# Autodesk Inventor assembly: scara 2.0
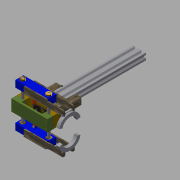
[picture p0: Inventor's stored thumbnail of the model, 180x180]
Saved by Autodesk Inventor 2019 (Build 230136000, 136)
## iProperties
Created: 2021-10-30
Part Number: scara 2.0
Document SubType Name: Assembly
Designer: Mohamed
Author: Mohamed
## Documents named in this file (21)
- F:\Semester 7\Design of mechatronics 1\SSCARA Robot\scara 2.0.iam
- F:\Semester 7\Design of mechatronics 1\SSCARA Robot\g_6mm rod.ipt
- F:\Semester 7\Design of mechatronics 1\SSCARA Robot\g_servo mount 1.ipt
- F:\Semester 7\Design of mechatronics 1\SSCARA Robot\g_servo mount 2.ipt
- F:\Semester 7\Design of mechatronics 1\SSCARA Robot\MG995.ipt
- F:\Semester 7\Design of mechatronics 1\SSCARA Robot\g_servo horn.ipt
- F:\Semester 7\Design of mechatronics 1\SSCARA Robot\g_connector x4.ipt
- F:\Semester 7\Design of mechatronics 1\SSCARA Robot\g_bolt.ipt
- F:\Semester 7\Design of mechatronics 1\SSCARA Robot\g_nut.ipt
- F:\Semester 7\Design of mechatronics 1\SSCARA Robot\g_griper side.ipt
- F:\Semester 7\Design of mechatronics 1\SSCARA Robot\g_griper side2.ipt
- F:\Semester 7\Design of mechatronics 1\SSCARA Robot\g_linear bearing 8mm.ipt
- F:\Semester 7\Design of mechatronics 1\SSCARA Robot\g_mount 1.ipt
- F:\Semester 7\Design of mechatronics 1\SSCARA Robot\g_mount 2.ipt
- F:\Semester 7\Design of mechatronics 1\SSCARA Robot\g_vslot 20x40.ipt
- F:\Semester 7\Design of mechatronics 1\SSCARA Robot\g_arm_v_1.ipt
- F:\Semester 7\Design of mechatronics 1\SSCARA Robot\g_arm_v_2.ipt
- F:\Semester 7\Design of mechatronics 1\SSCARA Robot\g_spacer_v.ipt
- F:\Semester 7\Design of mechatronics 1\SSCARA Robot\g_arm_v_3.ipt
- F:\Semester 7\Design of mechatronics 1\SSCARA Robot\g_griper left jaw_arm.ipt
- F:\Semester 7\Design of mechatronics 1\SSCARA Robot\g_jaws.ipt
## Components (42 placed, 20 different names)
1. g_6mm rod:1 — Mate:19, Flush:5, Mate:21, Mate:37
2. g_servo mount 1:1 — Mate:1, Mate:2, Mate:3, Flush:4, Mate:19, Flush:5, Mate:20, Flush:6, Mate:32, Flush:11, Flush:12, Mate:38, Mate:39, Mate:40, Mate:41, Mate:42, Mate:43, Mate:44, Mate:46, Mate:64
3. g_servo mount 2:1 — Mate:32, Flush:11, Flush:12
4. MG995:1 — Mate:1, Mate:2, Mate:3, Mate:4, Flush:1, Flush:4
5. g_servo horn:1 — Mate:4, Flush:1, Mate:5, Mate:6, Mate:7, Mate:8, Mate:9, Mate:10, Mate:11, Mate:12, Mate:14, Mate:16
6. g_connector x4:1 — Mate:5, Mate:6, Mate:13, Flush:8
7. g_connector x4:2 — Mate:7, Mate:8, Flush:8, Mate:24, Mate:25, Mate:26, Mate:27
8. g_connector x4:3 — Mate:9, Mate:10, Flush:7, Mate:23, Mate:28, Mate:29
9. g_connector x4:4 — Mate:11, Mate:12, Mate:15, Flush:7
10. g_bolt:1 — Mate:26, Mate:27, Mate:30, Flush:9
11. g_bolt:2 — Mate:15, Mate:16, Mate:18, Flush:3
12. g_bolt:3 — Mate:28, Mate:29, Mate:31, Flush:10
13. g_bolt:4 — Mate:13, Mate:14, Mate:17, Flush:2
14. g_nut:1 — Mate:30, Flush:9
15. g_nut:2 — Mate:31, Flush:10
16. g_nut:3 — Mate:18, Flush:3
17. g_nut:4 — Mate:17, Flush:2
18. g_griper side:1 — Mate:21, Mate:22, Mate:23, Mate:35, Flush:15, Mate:36, Flush:16, Mate:71, Mate:72, Mate:73, Mate:74, Mate:75, Mate:76
19. g_6mm rod:2 — Mate:20, Flush:6, Mate:22
20. g_griper side2:1 — Mate:24, Mate:25, Mate:33, Flush:13, Mate:34, Flush:14, Mate:65, Mate:66, Mate:67, Mate:68, Mate:69, Mate:70
21. g_linear bearing 8mm:1 — Mate:35, Flush:15
22. g_linear bearing 8mm:2 — Mate:33, Flush:13, Mate:37
23. g_linear bearing 8mm:3 — Mate:36, Flush:16
24. g_linear bearing 8mm:4 — Mate:34, Flush:14
25. g_mount 1:1 — Mate:38, Mate:39, Mate:40, Mate:45, Flush:17
26. g_mount 2:1 — Mate:41, Mate:42, Mate:43, Flush:18, Flush:19
27. g_vslot 20x40:1 — Mate:50, Mate:51, Mate:52
28. g_arm_v_1:1 — Mate:44, Mate:45, Flush:17, Mate:47, Mate:48, Mate:49, Mate:56, Mate:57, Mate:58, Flush:22, Mate:63, Flush:25
29. g_arm_v_1:2 — Mate:46, Flush:18, Flush:19, Mate:62, Flush:20, Flush:21
30. g_arm_v_2:1 — Mate:47, Mate:48, Mate:49, Mate:50, Mate:51, Mate:52, Flush:23, Flush:24
31. g_spacer_v:1 — Mate:59, Mate:60, Mate:61, Mate:62, Flush:20, Flush:21
32. g_spacer_v:2 — Mate:59, Mate:60, Mate:61
33. g_spacer_v:3 — Mate:53, Mate:54, Mate:55, Mate:57
34. g_spacer_v:4 — Mate:53, Mate:54, Mate:55, Mate:56, Mate:58
35. g_arm_v_3:1 — Flush:22, Flush:23, Flush:24
36. g_arm_v_3:2 — Mate:63, Mate:64, Flush:25
37. g_griper left jaw_arm:1 — Mate:65, Mate:66, Mate:67, Mate:77, Mate:78, Flush:26
38. g_griper left jaw_arm:2 — Mate:68, Mate:69, Mate:70
39. g_griper left jaw_arm:3 — Mate:71, Mate:72, Mate:73, Mate:79, Flush:27, Mate:80
40. g_griper left jaw_arm:4 — Mate:74, Mate:75, Mate:76
41. g_jaws:1 — Mate:77, Mate:78, Flush:26
42. g_jaws:2 — Mate:79, Flush:27, Mate:80
## Relationships (107: Mate 80, Flush 27)
- Mate:1 (0.5 mm): g_servo mount 1:1 ↔ MG995:1
- Mate:2 (0.5 mm): g_servo mount 1:1 ↔ MG995:1
- Mate:3: g_servo mount 1:1 ↔ MG995:1
- Mate:4: MG995:1 ↔ g_servo horn:1
- Flush:1 (-0.5 mm): MG995:1 ↔ g_servo horn:1
- Mate:5: g_servo horn:1 ↔ g_connector x4:1
- Mate:6: g_servo horn:1 ↔ g_connector x4:1
- Mate:7: g_servo horn:1 ↔ g_connector x4:2
- Mate:8: g_servo horn:1 ↔ g_connector x4:2
- Mate:9: g_servo horn:1 ↔ g_connector x4:3
- Mate:10: g_servo horn:1 ↔ g_connector x4:3
- Mate:11: g_servo horn:1 ↔ g_connector x4:4
- Mate:12: g_servo horn:1 ↔ g_connector x4:4
- Mate:13: g_connector x4:1 ↔ g_bolt:4
- Mate:14: g_servo horn:1 ↔ g_bolt:4
- Mate:15: g_connector x4:4 ↔ g_bolt:2
- Mate:16: g_servo horn:1 ↔ g_bolt:2
- Mate:17: g_bolt:4 ↔ g_nut:4
- Flush:2: g_bolt:4 ↔ g_nut:4
- Mate:18: g_bolt:2 ↔ g_nut:3
- Flush:3: g_bolt:2 ↔ g_nut:3
- Flush:4 (-1 mm): g_servo mount 1:1 ↔ MG995:1
- Mate:19: g_6mm rod:1 ↔ g_servo mount 1:1
- Flush:5 (-52.5 mm): g_6mm rod:1 ↔ g_servo mount 1:1
- Mate:20: g_servo mount 1:1 ↔ g_6mm rod:2
- Flush:6 (-52.5 mm): g_servo mount 1:1 ↔ g_6mm rod:2
- Mate:21: g_6mm rod:1 ↔ g_griper side:1
- Mate:22: g_griper side:1 ↔ g_6mm rod:2
- Flush:7: g_connector x4:3 ↔ g_connector x4:4
- Flush:8: g_connector x4:1 ↔ g_connector x4:2
- Mate:23: g_connector x4:3 ↔ g_griper side:1
- Mate:24: g_connector x4:2 ↔ g_griper side2:1
- Mate:25: g_connector x4:2 ↔ g_griper side2:1
- Mate:26: g_connector x4:2 ↔ g_bolt:1
- Mate:27: g_connector x4:2 ↔ g_bolt:1
- Mate:28: g_connector x4:3 ↔ g_bolt:3
- Mate:29: g_connector x4:3 ↔ g_bolt:3
- Mate:30: g_bolt:1 ↔ g_nut:1
- Flush:9: g_bolt:1 ↔ g_nut:1
- Mate:31: g_bolt:3 ↔ g_nut:2
- Flush:10: g_bolt:3 ↔ g_nut:2
- Mate:32: g_servo mount 1:1 ↔ g_servo mount 2:1
- Flush:11: g_servo mount 1:1 ↔ g_servo mount 2:1
- Flush:12: g_servo mount 1:1 ↔ g_servo mount 2:1
- Mate:33: g_griper side2:1 ↔ g_linear bearing 8mm:2
- Flush:13: g_griper side2:1 ↔ g_linear bearing 8mm:2
- Mate:34: g_griper side2:1 ↔ g_linear bearing 8mm:4
- Flush:14: g_griper side2:1 ↔ g_linear bearing 8mm:4
- Mate:35: g_griper side:1 ↔ g_linear bearing 8mm:1
- Flush:15: g_griper side:1 ↔ g_linear bearing 8mm:1
- Mate:36: g_griper side:1 ↔ g_linear bearing 8mm:3
- Flush:16: g_griper side:1 ↔ g_linear bearing 8mm:3
- Mate:37: g_6mm rod:1 ↔ g_linear bearing 8mm:2
- Mate:38: g_servo mount 1:1 ↔ g_mount 1:1
- Mate:39: g_servo mount 1:1 ↔ g_mount 1:1
- Mate:40: g_servo mount 1:1 ↔ g_mount 1:1
- Mate:41: g_servo mount 1:1 ↔ g_mount 2:1
- Mate:42: g_servo mount 1:1 ↔ g_mount 2:1
- Mate:43: g_servo mount 1:1 ↔ g_mount 2:1
- Mate:44: g_servo mount 1:1 ↔ g_arm_v_1:1
- Mate:45: g_mount 1:1 ↔ g_arm_v_1:1
- Flush:17: g_mount 1:1 ↔ g_arm_v_1:1
- Mate:46: g_servo mount 1:1 ↔ g_arm_v_1:2
- Flush:18: g_mount 2:1 ↔ g_arm_v_1:2
- Flush:19: g_mount 2:1 ↔ g_arm_v_1:2
- Mate:47: g_arm_v_1:1 ↔ g_arm_v_2:1
- Mate:48: g_arm_v_1:1 ↔ g_arm_v_2:1
- Mate:49: g_arm_v_1:1 ↔ g_arm_v_2:1
- Mate:50: g_vslot 20x40:1 ↔ g_arm_v_2:1
- Mate:51: g_vslot 20x40:1 ↔ g_arm_v_2:1
- Mate:52: g_vslot 20x40:1 ↔ g_arm_v_2:1
- Mate:53: g_spacer_v:3 ↔ g_spacer_v:4
- Mate:54: g_spacer_v:3 ↔ g_spacer_v:4
- Mate:55: g_spacer_v:3 ↔ g_spacer_v:4
- Mate:56: g_arm_v_1:1 ↔ g_spacer_v:4
- Mate:57: g_arm_v_1:1 ↔ g_spacer_v:3
- Mate:58: g_arm_v_1:1 ↔ g_spacer_v:4
- Mate:59: g_spacer_v:1 ↔ g_spacer_v:2
- Mate:60: g_spacer_v:1 ↔ g_spacer_v:2
- Mate:61: g_spacer_v:1 ↔ g_spacer_v:2
- Mate:62: g_arm_v_1:2 ↔ g_spacer_v:1
- Flush:20: g_arm_v_1:2 ↔ g_spacer_v:1
- Flush:21: g_arm_v_1:2 ↔ g_spacer_v:1
- Flush:22: g_arm_v_1:1 ↔ g_arm_v_3:1
- Flush:23: g_arm_v_2:1 ↔ g_arm_v_3:1
- Flush:24: g_arm_v_2:1 ↔ g_arm_v_3:1
- Mate:63: g_arm_v_1:1 ↔ g_arm_v_3:2
- Mate:64: g_servo mount 1:1 ↔ g_arm_v_3:2
- Flush:25: g_arm_v_1:1 ↔ g_arm_v_3:2
- Mate:65: g_griper side2:1 ↔ g_griper left jaw_arm:1
- Mate:66: g_griper side2:1 ↔ g_griper left jaw_arm:1
- Mate:67: g_griper side2:1 ↔ g_griper left jaw_arm:1
- Mate:68: g_griper side2:1 ↔ g_griper left jaw_arm:2
- Mate:69: g_griper side2:1 ↔ g_griper left jaw_arm:2
- Mate:70: g_griper side2:1 ↔ g_griper left jaw_arm:2
- Mate:71: g_griper side:1 ↔ g_griper left jaw_arm:3
- Mate:72: g_griper side:1 ↔ g_griper left jaw_arm:3
- Mate:73: g_griper side:1 ↔ g_griper left jaw_arm:3
- Mate:74: g_griper side:1 ↔ g_griper left jaw_arm:4
- Mate:75: g_griper side:1 ↔ g_griper left jaw_arm:4
- Mate:76: g_griper side:1 ↔ g_griper left jaw_arm:4
- Mate:77: g_griper left jaw_arm:1 ↔ g_jaws:1
- Mate:78: g_griper left jaw_arm:1 ↔ g_jaws:1
- Flush:26: g_griper left jaw_arm:1 ↔ g_jaws:1
- Mate:79: g_griper left jaw_arm:3 ↔ g_jaws:2
- Flush:27: g_griper left jaw_arm:3 ↔ g_jaws:2
- Mate:80: g_griper left jaw_arm:3 ↔ g_jaws:2
